# Autodesk Inventor assembly: Finger Assembly
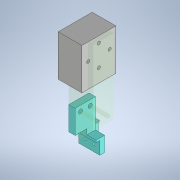
[picture p0: Inventor's stored thumbnail of the model, 180x180]
Saved by Autodesk Inventor 2022 (Build 260153000, 153)
## iProperties
Created: 2021-09-24
Part Number: Finger Assembly
Document SubType Name: Assembly
Designer: kylem
Author: kylem
## Documents named in this file (4)
- C:\Users\kylem\OneDrive\Documents\1 - Documents\Gripper Design\Finger Assembly.iam
- C:\Users\kylem\OneDrive\Documents\1 - Documents\Gripper Design\Finger.ipt
- C:\Users\kylem\OneDrive\Documents\1 - Documents\Gripper Design\Finger_mount.ipt
- C:\Users\kylem\OneDrive\Documents\1 - Documents\Gripper Design\Contactile Sensor.ipt
## Components (3 placed, 3 different names)
1. Finger:1 — Mate:1, Mate:2, Flush:1, Mate:3
2. Finger_mount:1 — Mate:1, Mate:2
3. Contactile Sensor:1 — Flush:1, Mate:3
## Relationships (4: Mate 3, Flush 1)
- Mate:1: Finger:1 ↔ Finger_mount:1
- Mate:2: Finger:1 ↔ Finger_mount:1
- Flush:1: Finger:1 ↔ Contactile Sensor:1
- Mate:3: Finger:1 ↔ Contactile Sensor:1
